# Autodesk Inventor assembly: ASM IMU
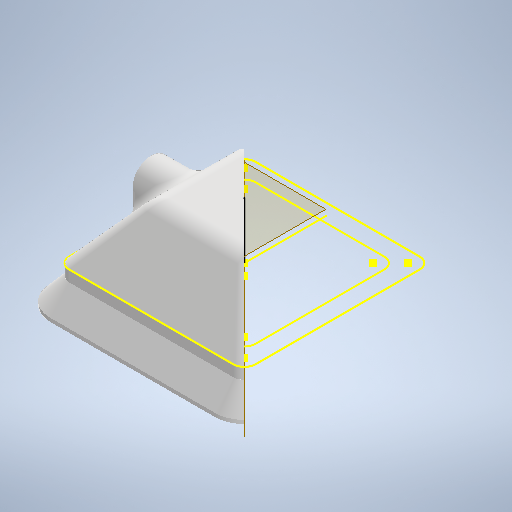
[picture p0: Inventor's stored thumbnail of the model, 512x512]
Saved by Autodesk Inventor 2025.2 (Build 292293000, 293)
## iProperties
Created: 2024-11-14
Part Number: ASM IMU
Document SubType Name: Assembly
Designer: matss
Author: matss
## Documents named in this file (5)
- C:\Users\tills\Desktop\3_Semester\Elective_Health_Device\Wearable-Health-Device\ASM IMU.iam
- C:\Users\tills\Desktop\3_Semester\Elective_Health_Device\Wearable-Health-Device\MPU6050 v2\MPU6050 v2\MPU6050 v2.ipt
- C:\Users\tills\Desktop\3_Semester\Elective_Health_Device\Wearable-Health-Device\IMU_Base_T-Shirt.ipt
- C:\Users\tills\Desktop\3_Semester\Elective_Health_Device\Wearable-Health-Device\IMU_mount_baseplate.ipt
- C:\Users\tills\Desktop\3_Semester\Elective_Health_Device\Wearable-Health-Device\IMU_mount_cover.ipt
## Components (4 placed, 4 different names)
1. MPU6050 v2:1 — Passend:8, Winkel:2, Passend:9
2. IMU_Base_T-Shirt:1 — Passend:1, Winkel:1, Passend:6, Passend:7, Passend:13, Passend:15
3. IMU_mount_baseplate:1 — Passend:6, Passend:7, Passend:8, Passend:9, Passend:13, Passend:14, Passend:16
4. IMU_mount_cover:1 — Passend:14, Passend:15, Passend:16
## Relationships (11: Mate 9, Angle 2)
- Passend:1 [Mate]: IMU_Base_T-Shirt:1
- Winkel:1 [Angle] (0 deg): IMU_Base_T-Shirt:1
- Passend:6 [Mate]: IMU_Base_T-Shirt:1 ↔ IMU_mount_baseplate:1
- Passend:7 [Mate]: IMU_Base_T-Shirt:1 ↔ IMU_mount_baseplate:1
- Passend:8 [Mate]: MPU6050 v2:1 ↔ IMU_mount_baseplate:1
- Winkel:2 [Angle] (90 deg): MPU6050 v2:1
- Passend:9 [Mate] (2 mm): MPU6050 v2:1 ↔ IMU_mount_baseplate:1
- Passend:13 [Mate]: IMU_Base_T-Shirt:1 ↔ IMU_mount_baseplate:1
- Passend:14 [Mate] (0.25 mm): IMU_mount_baseplate:1 ↔ IMU_mount_cover:1
- Passend:15 [Mate]: IMU_Base_T-Shirt:1 ↔ IMU_mount_cover:1
- Passend:16 [Mate] (0.25 mm): IMU_mount_baseplate:1 ↔ IMU_mount_cover:1
